# Autodesk Inventor assembly: Battery_Pack
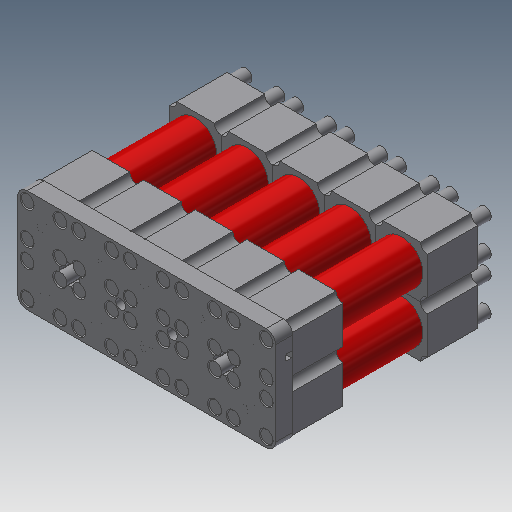
[picture p0: Inventor's stored thumbnail of the model, 512x512]
Saved by Autodesk Inventor 2018 (Build 220112000, 112)
## iProperties
Created: 2019-09-04
Part Number: Battery_Pack
Document SubType Name: Assembly
Designer: Clevo
Author: Clevo
## Documents named in this file (4)
- E:\Hardware_Accelerated_Robot\Hardware\Battery\Battery_Pack.iam
- E:\Hardware_Accelerated_Robot\Hardware\Battery\Battery_Module.iam
- E:\Hardware_Accelerated_Robot\Hardware\Screws\90592A085_STEEL HEX NUT.ipt
- E:\Hardware_Accelerated_Robot\Hardware\CustomParts\Battery_Cover.ipt
## Components (21 placed, 3 different names)
1. Battery_Module:1 [sub-assembly] — Mate:1, Flush:1, Flush:2, Mate:2, Flush:3, Flush:4, Mate:9, Flush:17, Mate:17, Mate:25
2. Battery_Module:2 [sub-assembly] — Mate:1, Flush:1, Flush:2, Mate:4, Flush:7, Flush:8, Mate:16, Mate:28
3. Battery_Module:3 [sub-assembly] — Mate:2, Flush:3, Flush:4, Mate:3, Flush:5, Flush:6, Mate:18, Mate:22
4. Battery_Module:4 [sub-assembly] — Mate:3, Flush:5, Flush:6, Mate:19, Mate:20, Flush:19, Flush:20, Mate:30
5. Battery_Module:5 [sub-assembly] — Mate:4, Flush:7, Flush:8, Flush:18, Mate:15, Mate:29
6. Battery_Module:6 [sub-assembly] — Mate:9, Flush:17, Mate:12, Mate:24
7. Battery_Module:7 [sub-assembly] — Mate:13, Mate:26
8. Battery_Module:8 [sub-assembly] — Mate:11, Mate:23
9. Battery_Module:9 [sub-assembly] — Mate:10, Mate:21
10. Battery_Module:10 [sub-assembly] — Flush:18, Mate:14, Mate:27
11. 90592A085_STEEL HEX NUT:1 — Mate:12, Mate:24
12. 90592A085_STEEL HEX NUT:2 — Mate:14, Mate:27
13. 90592A085_STEEL HEX NUT:3 — Mate:17, Mate:25
14. 90592A085_STEEL HEX NUT:4 — Mate:18, Mate:22
15. 90592A085_STEEL HEX NUT:5 — Mate:15, Mate:29
16. 90592A085_STEEL HEX NUT:6 — Mate:16, Mate:28
17. 90592A085_STEEL HEX NUT:7 — Mate:19, Mate:20
18. 90592A085_STEEL HEX NUT:8 — Mate:13, Mate:26
19. 90592A085_STEEL HEX NUT:9 — Mate:11, Mate:23
20. 90592A085_STEEL HEX NUT:10 — Mate:10, Mate:21
21. Battery_Cover:1 — Flush:19, Flush:20, Mate:30
## Relationships (50: Mate 30, Flush 20)
- Mate:1: Battery_Module:1 ↔ Battery_Module:2
- Flush:1: Battery_Module:1 ↔ Battery_Module:2
- Flush:2: Battery_Module:1 ↔ Battery_Module:2
- Mate:2: Battery_Module:1 ↔ Battery_Module:3
- Flush:3: Battery_Module:1 ↔ Battery_Module:3
- Flush:4: Battery_Module:1 ↔ Battery_Module:3
- Mate:3: Battery_Module:3 ↔ Battery_Module:4
- Flush:5: Battery_Module:3 ↔ Battery_Module:4
- Flush:6: Battery_Module:3 ↔ Battery_Module:4
- Mate:4: Battery_Module:2 ↔ Battery_Module:5
- Flush:7: Battery_Module:2 ↔ Battery_Module:5
- Flush:8: Battery_Module:2 ↔ Battery_Module:5
- [Mate]: Battery_Module:6 ↔ Battery_Module:7
- [Flush]: Battery_Module:6 ↔ Battery_Module:7
- [Flush]: Battery_Module:6 ↔ Battery_Module:7
- [Mate]: Battery_Module:6 ↔ Battery_Module:8
- [Flush]: Battery_Module:6 ↔ Battery_Module:8
- [Flush]: Battery_Module:6 ↔ Battery_Module:8
- [Mate]: Battery_Module:8 ↔ Battery_Module:9
- [Flush]: Battery_Module:8 ↔ Battery_Module:9
- [Flush]: Battery_Module:8 ↔ Battery_Module:9
- [Mate]: Battery_Module:7 ↔ Battery_Module:10
- [Flush]: Battery_Module:7 ↔ Battery_Module:10
- [Flush]: Battery_Module:7 ↔ Battery_Module:10
- Mate:9: Battery_Module:1 ↔ Battery_Module:6
- Flush:17: Battery_Module:1 ↔ Battery_Module:6
- Flush:18: Battery_Module:5 ↔ Battery_Module:10
- Mate:10: Battery_Module:9 ↔ 90592A085_STEEL HEX NUT:10
- Mate:11: Battery_Module:8 ↔ 90592A085_STEEL HEX NUT:9
- Mate:12: Battery_Module:6 ↔ 90592A085_STEEL HEX NUT:1
- Mate:13: Battery_Module:7 ↔ 90592A085_STEEL HEX NUT:8
- Mate:14: Battery_Module:10 ↔ 90592A085_STEEL HEX NUT:2
- Mate:15: Battery_Module:5 ↔ 90592A085_STEEL HEX NUT:5
- Mate:16: Battery_Module:2 ↔ 90592A085_STEEL HEX NUT:6
- Mate:17: Battery_Module:1 ↔ 90592A085_STEEL HEX NUT:3
- Mate:18: Battery_Module:3 ↔ 90592A085_STEEL HEX NUT:4
- Mate:19: Battery_Module:4 ↔ 90592A085_STEEL HEX NUT:7
- Mate:20 (1.5 mm): Battery_Module:4 ↔ 90592A085_STEEL HEX NUT:7
- Mate:21 (1.5 mm): Battery_Module:9 ↔ 90592A085_STEEL HEX NUT:10
- Mate:22 (1.5 mm): Battery_Module:3 ↔ 90592A085_STEEL HEX NUT:4
- Mate:23 (1.5 mm): Battery_Module:8 ↔ 90592A085_STEEL HEX NUT:9
- Mate:24 (1.5 mm): Battery_Module:6 ↔ 90592A085_STEEL HEX NUT:1
- Mate:25 (1.5 mm): Battery_Module:1 ↔ 90592A085_STEEL HEX NUT:3
- Mate:26 (1.5 mm): Battery_Module:7 ↔ 90592A085_STEEL HEX NUT:8
- Mate:27 (1.5 mm): Battery_Module:10 ↔ 90592A085_STEEL HEX NUT:2
- Mate:28 (1.5 mm): Battery_Module:2 ↔ 90592A085_STEEL HEX NUT:6
- Mate:29 (1.5 mm): Battery_Module:5 ↔ 90592A085_STEEL HEX NUT:5
- Flush:19: Battery_Module:4 ↔ Battery_Cover:1
- Flush:20: Battery_Module:4 ↔ Battery_Cover:1
- Mate:30: Battery_Module:4 ↔ Battery_Cover:1
## Named parameters: d12_d10 = 0 mm, d13_d11 = 0 mm, d14_d1 = 0 mm, d15_d2 = 0 mm, d16_d3 = 0 mm, d17_d4 = 0 mm, d18_d5 = 0 mm, d19_d6 = 0 mm, d20_d7 = 0 mm, d21_d8 = 0 mm, d22_d9 = 0 mm, d23_d0 = 0 mm
